# Autodesk Inventor assembly: Höhenverstellung-2
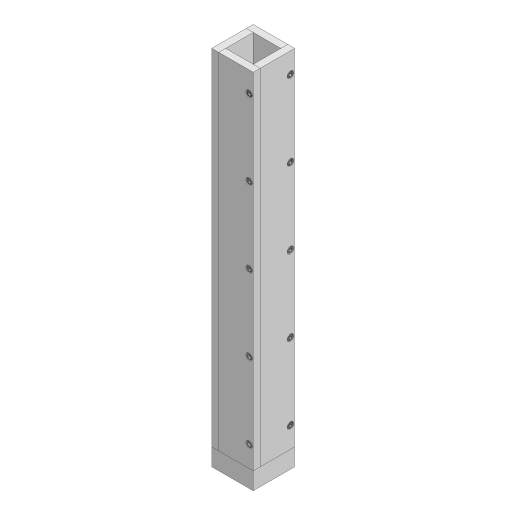
[picture p0: Inventor's stored thumbnail of the model, 512x512]
Saved by Autodesk Inventor 2024.3 (Build 283343000, 343)
## iProperties
Created: 2025-05-16
Part Number: Höhenverstellung-2
Document SubType Name: Assembly
Designer: Demir
Author: Demir
## Documents named in this file (7)
- Z:\Verfahreinheit-SWB\Vincent\Höhenverstellung-2.iam
- Z:\Verfahreinheit-SWB\Vincent\Platte-2.ipt
- Z:\Verfahreinheit-SWB\Vincent\Platte-1.ipt
- C:\InventorNormteile\Content Center\Libraries\de-DE\DIN 912\DIN 912 - M8 x 1,25 x 25 x 21,875.ipt
- C:\InventorNormteile\Content Center\Libraries\de-DE\DIN 912\DIN 912 - M5 x 0,8 x 16 x 14.ipt
- C:\InventorNormteile\Content Center\Libraries\de-DE\DIN 912\DIN 912 - M5 x 0,8 x 30 x 22.ipt
- Z:\Verfahreinheit-SWB\Vincent\Deckel-2.ipt
## Components (31 placed, 6 different names)
1. Platte-2:1 — Passend:1, Fluchtend:1, Fluchtend:2, Passend:4, Fluchtend:8, Fluchtend:13, Passend:9, Fluchtend:14, Einfügen:27
2. Platte-1:1 — Passend:1, Fluchtend:1, Fluchtend:2, Einfügen:21, Einfügen:22, Passend:7, Fluchtend:10, Fluchtend:12, Einfügen:26
3. Deckel-2:1 — Passend:4, Fluchtend:8, Einfügen:30, Einfügen:31, Einfügen:32, Einfügen:33
4. DIN 912 - ersetzt durch DIN EN ISO 4762 M8 x 25:1 — Einfügen:21
5. DIN 912 - ersetzt durch DIN EN ISO 4762 M8 x 25:2 — Einfügen:22
6. Platte-2:2 — Passend:7, Fluchtend:10, Fluchtend:12, Passend:8, Einfügen:29
7. Platte-2:3 — Passend:8, Fluchtend:13, Passend:9, Fluchtend:14, Einfügen:28
8. DIN 912 - ersetzt durch DIN EN ISO 4762 M5 x 16:21 — Einfügen:30
9. DIN 912 - ersetzt durch DIN EN ISO 4762 M5 x 16:22 — Einfügen:31
10. DIN 912 - ersetzt durch DIN EN ISO 4762 M5 x 30:1 — Einfügen:32
11. DIN 912 - ersetzt durch DIN EN ISO 4762 M5 x 16:24 — Einfügen:33
12. DIN 912 - ersetzt durch DIN EN ISO 4762 M5 x 16:1 — Einfügen:27
13. DIN 912 - ersetzt durch DIN EN ISO 4762 M5 x 16:2
14. DIN 912 - ersetzt durch DIN EN ISO 4762 M5 x 16:3
15. DIN 912 - ersetzt durch DIN EN ISO 4762 M5 x 16:4
16. DIN 912 - ersetzt durch DIN EN ISO 4762 M5 x 16:5
17. DIN 912 - ersetzt durch DIN EN ISO 4762 M5 x 16:6 — Einfügen:26
18. DIN 912 - ersetzt durch DIN EN ISO 4762 M5 x 16:7 — Einfügen:29
19. DIN 912 - ersetzt durch DIN EN ISO 4762 M5 x 16:8 — Einfügen:28
20. DIN 912 - ersetzt durch DIN EN ISO 4762 M5 x 16:9
21. DIN 912 - ersetzt durch DIN EN ISO 4762 M5 x 16:10
22. DIN 912 - ersetzt durch DIN EN ISO 4762 M5 x 16:11
23. DIN 912 - ersetzt durch DIN EN ISO 4762 M5 x 16:12
24. DIN 912 - ersetzt durch DIN EN ISO 4762 M5 x 16:13
25. DIN 912 - ersetzt durch DIN EN ISO 4762 M5 x 16:14
26. DIN 912 - ersetzt durch DIN EN ISO 4762 M5 x 16:15
27. DIN 912 - ersetzt durch DIN EN ISO 4762 M5 x 16:16
28. DIN 912 - ersetzt durch DIN EN ISO 4762 M5 x 16:17
29. DIN 912 - ersetzt durch DIN EN ISO 4762 M5 x 16:18
30. DIN 912 - ersetzt durch DIN EN ISO 4762 M5 x 16:19
31. DIN 912 - ersetzt durch DIN EN ISO 4762 M5 x 16:20
## Component patterns: (5 elements, first: DIN 912 - ersetzt durch DIN EN ISO 4762 M5 x 16:1), (5 elements, first: DIN 912 - ersetzt durch DIN EN ISO 4762 M5 x 16:6 + DIN 912 - ersetzt durch DIN EN ISO 4762 M5 x 16:7 + DIN 912 - ersetzt durch DIN EN ISO 4762 M5 x 16:8)
## Relationships (22: Insert 10, Flush 7, Mate 5)
- Passend:1 [Mate]: Platte-2:1 ↔ Platte-1:1
- Fluchtend:1 [Flush]: Platte-2:1 ↔ Platte-1:1
- Fluchtend:2 [Flush]: Platte-2:1 ↔ Platte-1:1
- Passend:4 [Mate]: Platte-2:1 ↔ Deckel-2:1
- Fluchtend:8 [Flush]: Platte-2:1 ↔ Deckel-2:1
- Einfügen:21 [Insert]: Platte-1:1 ↔ DIN 912 - ersetzt durch DIN EN ISO 4762 M8 x 25:1
- Einfügen:22 [Insert]: Platte-1:1 ↔ DIN 912 - ersetzt durch DIN EN ISO 4762 M8 x 25:2
- Passend:7 [Mate]: Platte-1:1 ↔ Platte-2:2
- Fluchtend:10 [Flush]: Platte-1:1 ↔ Platte-2:2
- Fluchtend:12 [Flush]: Platte-1:1 ↔ Platte-2:2
- Passend:8 [Mate]: Platte-2:2 ↔ Platte-2:3
- Fluchtend:13 [Flush]: Platte-2:1 ↔ Platte-2:3
- Passend:9 [Mate]: Platte-2:1 ↔ Platte-2:3
- Fluchtend:14 [Flush]: Platte-2:1 ↔ Platte-2:3
- Einfügen:26 [Insert]: Platte-1:1 ↔ DIN 912 - ersetzt durch DIN EN ISO 4762 M5 x 16:6
- Einfügen:27 [Insert]: Platte-2:1 ↔ DIN 912 - ersetzt durch DIN EN ISO 4762 M5 x 16:1
- Einfügen:28 [Insert]: Platte-2:3 ↔ DIN 912 - ersetzt durch DIN EN ISO 4762 M5 x 16:8
- Einfügen:29 [Insert]: Platte-2:2 ↔ DIN 912 - ersetzt durch DIN EN ISO 4762 M5 x 16:7
- Einfügen:30 [Insert]: Deckel-2:1 ↔ DIN 912 - ersetzt durch DIN EN ISO 4762 M5 x 16:21
- Einfügen:31 [Insert]: Deckel-2:1 ↔ DIN 912 - ersetzt durch DIN EN ISO 4762 M5 x 16:22
- Einfügen:32 [Insert]: Deckel-2:1 ↔ DIN 912 - ersetzt durch DIN EN ISO 4762 M5 x 30:1
- Einfügen:33 [Insert]: Deckel-2:1 ↔ DIN 912 - ersetzt durch DIN EN ISO 4762 M5 x 16:24
